# Autodesk Inventor assembly: rod_stand
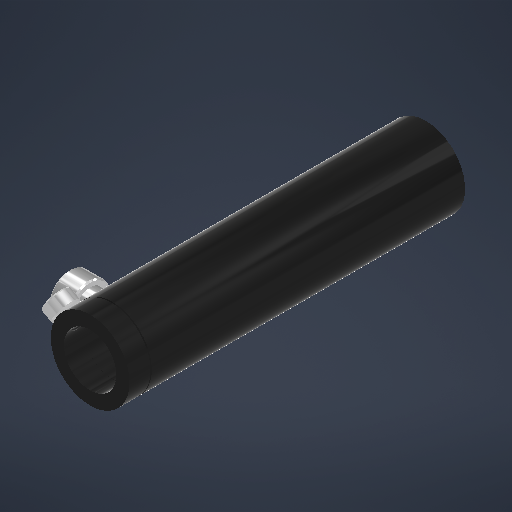
[picture p0: Inventor's stored thumbnail of the model, 512x512]
Saved by Autodesk Inventor 2026 (Build 300175050, 175E)
## iProperties
Created: 2025-07-09
Part Number: rod_stand
Document SubType Name: Assembly
Designer: jin20
Author: jin20
## Documents named in this file (5)
- C:\Users\jin20\Documents\装置CAD\RamanSystem\Stage\rod_stand\rod_stand.iam
- C:\Users\jin20\Documents\装置CAD\RamanSystem\Stage\rod_stand\stand_base.ipt
- C:\Users\jin20\Documents\装置CAD\RamanSystem\Stage\rod_stand\stand_handle.ipt
- C:\Users\jin20\Documents\装置CAD\RamanSystem\Stage\rod_stand\ring_base.ipt
- C:\Users\jin20\Documents\装置CAD\RamanSystem\Stage\rod_stand\ring_handle.ipt
## Components (4 placed, 4 different names)
1. stand_base:1 — リジッド:2, 回転:1
2. stand_handle:1 — リジッド:2
3. ring_base:1 — リジッド:1, 回転:1
4. ring_handle:1 — リジッド:1
## Relationships (3: WeldJoint 2, RevoluteJoint 1)
- リジッド:1 [WeldJoint]: ring_base:1 ↔ ring_handle:1
- リジッド:2 [WeldJoint]: stand_base:1 ↔ stand_handle:1
- 回転:1 [RevoluteJoint]: stand_base:1 ↔ ring_base:1
